# Autodesk Inventor assembly: The_Assembly
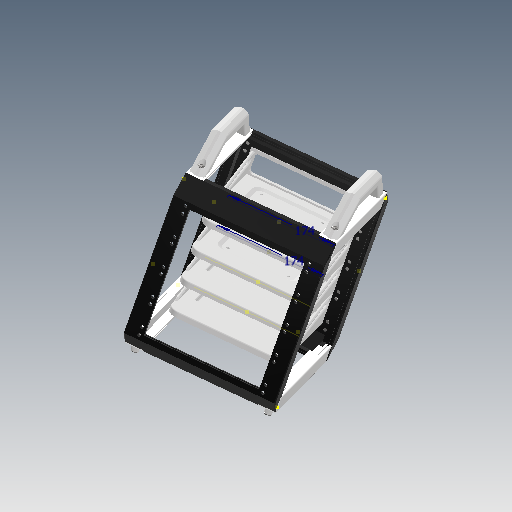
[picture p0: Inventor's stored thumbnail of the model, 512x512]
Saved by Autodesk Inventor 2027 (Build 310192060, 192F)
## iProperties
Created: 2026-07-27
Part Number: The_Assembly
Document SubType Name: Assembly
Designer: prest
Author: prest
## Documents named in this file (24)
- C:\Users\prest\OneDrive\Documents\Projects\Home_Lab_Rack\The_Assembly.iam
- C:\Users\prest\OneDrive\Documents\Projects\Home_Lab_Rack\Strut_Angled.ipt
- C:\Users\prest\OneDrive\Documents\Projects\Home_Lab_Rack\bottom_edge.ipt
- C:\Users\prest\OneDrive\Documents\Projects\Home_Lab_Rack\Strut_Horizontal.ipt
- C:\Users\prest\OneDrive\Documents\Inventor\Content Center Files\R2027\en-US\ANSI B18.3.4M(1)\ANSI B18.3.4M - M6 x 1 x 8(2).ipt
- C:\Users\prest\OneDrive\Documents\Projects\Home_Lab_Rack\mini_PC_mount.ipt
- C:\Users\prest\OneDrive\Documents\Projects\Home_Lab_Rack\router_mount.ipt
- C:\Users\prest\OneDrive\Documents\Projects\Home_Lab_Rack\side_panel_actual.ipt
- C:\Users\prest\OneDrive\Documents\Projects\Home_Lab_Rack\bottom_panel.ipt
- C:\Users\prest\OneDrive\Documents\Projects\Home_Lab_Rack\front_panel_mount_end.ipt
- C:\Users\prest\OneDrive\Documents\Projects\Home_Lab_Rack\top panel.ipt
- C:\Users\prest\OneDrive\Documents\Projects\Home_Lab_Rack\feet.ipt
- C:\Users\prest\OneDrive\Documents\Projects\Home_Lab_Rack\top_edge.ipt
- C:\Users\prest\OneDrive\Documents\Inventor\Content Center Files\R2027\en-US\ASME ANSI B18.3.5M(2)\ASME_ANSI B18.3.5M - M6x20(2).ipt
- C:\Users\prest\OneDrive\Documents\Projects\Home_Lab_Rack\Handle.ipt
- C:\Users\prest\OneDrive\Documents\Inventor\Content Center Files\R2027\en-US\ANSI B18.3.4M(1)\ANSI B18.3.4M - M6 x 1 x 16(2).ipt
- C:\Users\prest\OneDrive\Documents\Projects\Home_Lab_Rack\cable_basket.ipt
- C:\Users\prest\OneDrive\Documents\Projects\Home_Lab_Rack\Strut_Horizonal_Top.ipt
- C:\Users\prest\OneDrive\Documents\Projects\Home_Lab_Rack\MISC\Handle.ipt
- C:\Users\prest\OneDrive\Documents\Projects\Home_Lab_Rack\MISC\Feet.ipt
- C:\Users\prest\OneDrive\Documents\Projects\Home_Lab_Rack\Mounts\Front_Panel_Breathers.ipt
- C:\Users\prest\OneDrive\Documents\Projects\Home_Lab_Rack\Mounts\mini_PC_mount.ipt
- C:\Users\prest\OneDrive\Documents\Projects\Home_Lab_Rack\Mounts\router_mount.ipt
- C:\Users\prest\OneDrive\Documents\Projects\Home_Lab_Rack\Strut_Horizonal_Bottom.ipt
## Components (90 placed, 20 different names)
1. Handle:3 — Rigid:21, Rigid:23, Rigid:26
2. Handle:4 — Rigid:22, Rigid:24, Rigid:25
3. Broached Hexagon Socket Button Head Cap Screw - Metric M6 x 1 x 16:1 — Rigid:23, Rotational:25
4. Broached Hexagon Socket Button Head Cap Screw - Metric M6 x 1 x 16:2 — Rigid:24, Rotational:26
5. Broached Hexagon Socket Button Head Cap Screw - Metric M6 x 1 x 16:3 — Rigid:25, Rotational:27
6. Broached Hexagon Socket Button Head Cap Screw - Metric M6 x 1 x 16:4 — Rigid:26, Rotational:24
7. cable_basket:1 — Rotational:22, Mate:30
8. cable_basket:2 — Rotational:23, Mate:31
9. Strut_Horizonal_Top:1 — Rigid:29, Rigid:30, Rigid:33
10. Strut_Horizonal_Top:2 — Rigid:31, Rigid:32
11. Handle:5 — Rigid:33, Rotational:24, Rotational:26
12. Handle:6 — Rigid:32, Rotational:25, Rotational:27
13. Feet:1 — Rigid:35, Rigid:40
14. Feet:2 — Rigid:36, Rotational:52
15. Feet:3 — Rigid:37, Rigid:39
16. Feet:4 — Rigid:38, Rotational:51
17. Front_Panel_Breathers:1 — Rotational:28, Mate:45, Rotational:39, Rotational:40
18. mini_PC_mount:3 — Mate:39, Mate:40, Mate:41, Rotational:35, Rotational:36, Rotational:43, Rotational:44
19. router_mount:3 — Mate:32, Mate:33, Mate:34, Rotational:31, Rotational:32, Rotational:47, Rotational:48
20. Front_Panel_Breathers:2 — Rotational:29, Mate:35, Rotational:30, Rotational:49
21. router_mount:4 — Mate:36, Mate:37, Mate:38, Rotational:33, Rotational:34, Rotational:45, Rotational:46
22. mini_PC_mount:4 — Mate:42, Mate:43, Mate:44, Rotational:37, Rotational:38, Rotational:41, Rotational:42
23. Broached Hexagon Socket Button Head Cap Screw - Metric M6 x 1 x 16:5 — Rotational:30
24. Broached Hexagon Socket Button Head Cap Screw - Metric M6 x 1 x 16:6 — Rotational:31
25. Broached Hexagon Socket Button Head Cap Screw - Metric M6 x 1 x 16:7 — Rotational:32
26. Broached Hexagon Socket Button Head Cap Screw - Metric M6 x 1 x 16:8 — Rotational:33
27. Broached Hexagon Socket Button Head Cap Screw - Metric M6 x 1 x 16:9 — Rotational:34
28. Broached Hexagon Socket Button Head Cap Screw - Metric M6 x 1 x 16:10 — Rotational:35
29. Broached Hexagon Socket Button Head Cap Screw - Metric M6 x 1 x 16:11 — Rotational:36
30. Broached Hexagon Socket Button Head Cap Screw - Metric M6 x 1 x 16:12 — Rotational:37
31. Broached Hexagon Socket Button Head Cap Screw - Metric M6 x 1 x 16:13 — Rotational:44
32. Broached Hexagon Socket Button Head Cap Screw - Metric M6 x 1 x 16:14 — Rotational:43
33. Broached Hexagon Socket Button Head Cap Screw - Metric M6 x 1 x 16:15 — Rotational:42
34. Broached Hexagon Socket Button Head Cap Screw - Metric M6 x 1 x 16:16 — Rotational:41
35. Broached Hexagon Socket Button Head Cap Screw - Metric M6 x 1 x 16:17 — Rotational:40
36. Broached Hexagon Socket Button Head Cap Screw - Metric M6 x 1 x 16:18 — Rotational:39
37. Broached Hexagon Socket Button Head Cap Screw - Metric M6 x 1 x 16:19 — Rotational:38
38. Broached Hexagon Socket Button Head Cap Screw - Metric M6 x 1 x 16:20 — Rotational:48
39. Broached Hexagon Socket Button Head Cap Screw - Metric M6 x 1 x 16:21 — Rotational:47
40. Broached Hexagon Socket Button Head Cap Screw - Metric M6 x 1 x 16:22 — Rotational:46
41. Broached Hexagon Socket Button Head Cap Screw - Metric M6 x 1 x 16:23 — Rotational:45
42. Broached Hexagon Socket Button Head Cap Screw - Metric M6 x 1 x 16:24 — Rotational:49
43. Strut_Horizonal_Bottom:1 — Rotational:50, Mate:46, Rigid:37, Rigid:38
44. Strut_Horizonal_Bottom:2 — Rigid:34, Rigid:35, Rigid:36
45. Broached Hexagon Socket Flat Countersunk Head Cap Screws - Metric M6x20:5 — Rotational:52
46. Broached Hexagon Socket Flat Countersunk Head Cap Screws - Metric M6x20:6 — Rotational:51
47. Broached Hexagon Socket Flat Countersunk Head Cap Screws - Metric M6x20:3 — Flush:3, Mate:25, Rigid:40
48. Broached Hexagon Socket Flat Countersunk Head Cap Screws - Metric M6x20:4 — Flush:2, Mate:26, Rigid:39
49. Broached Hexagon Socket Button Head Cap Screw - Metric M6 x 1 x 8:1 — Rotational:1
50. Broached Hexagon Socket Button Head Cap Screw - Metric M6 x 1 x 8:2 — Rotational:2
51. Broached Hexagon Socket Button Head Cap Screw - Metric M6 x 1 x 8:3 — Rotational:3
52. Broached Hexagon Socket Button Head Cap Screw - Metric M6 x 1 x 8:4 — Rotational:5
53. Broached Hexagon Socket Button Head Cap Screw - Metric M6 x 1 x 8:5 — Rotational:6
54. Broached Hexagon Socket Button Head Cap Screw - Metric M6 x 1 x 8:6 — Rotational:4
55. Broached Hexagon Socket Button Head Cap Screw - Metric M6 x 1 x 8:7 — Rotational:7
56. Broached Hexagon Socket Button Head Cap Screw - Metric M6 x 1 x 8:8 — Rotational:8
57. Broached Hexagon Socket Button Head Cap Screw - Metric M6 x 1 x 8:13 — Rotational:14
58. Broached Hexagon Socket Button Head Cap Screw - Metric M6 x 1 x 8:14 — Rotational:15
59. Broached Hexagon Socket Button Head Cap Screw - Metric M6 x 1 x 8:15 — Rotational:16
60. Broached Hexagon Socket Button Head Cap Screw - Metric M6 x 1 x 8:17 — Rotational:17
61. Broached Hexagon Socket Button Head Cap Screw - Metric M6 x 1 x 8:18 — Rotational:19
62. Broached Hexagon Socket Button Head Cap Screw - Metric M6 x 1 x 8:19 — Rotational:18
63. Broached Hexagon Socket Button Head Cap Screw - Metric M6 x 1 x 8:20 — Rotational:20
64. Broached Hexagon Socket Button Head Cap Screw - Metric M6 x 1 x 8:21 — Rotational:21
65. Strut_Angled:1 — Rigid:9, Rotational:15, Rotational:16, Rotational:18, Rotational:19, Mate:13, Rigid:16, Mate:19, Mate:20, Mate:22, Mate:24, Rigid:30, Rigid:31
66. Strut_Angled:2 — Rigid:10, Rotational:14, Rotational:17, Rotational:20, Rotational:21, Mate:21, Mate:23, Rigid:29
67. Strut_Angled:3 — Rigid:3, Rigid:4, Rigid:5, Rotational:1, Rotational:2, Rotational:5, Rotational:6, Mate:46, Rigid:34
68. Strut_Angled:4 — Rigid:1, Rigid:2, Rigid:6, Rigid:7, Rotational:3, Rotational:4, Rotational:7, Rotational:8, Mate:16, Rotational:50
69. Strut_Horizontal:1 — Rigid:7, Rigid:9, Mate:1, Mate:2, Mate:4, Mate:5, Mate:8, Mate:11, Mate:14, Mate:17, Rotational:28, Mate:34, Mate:35, Mate:36, Mate:38, Mate:39, Mate:43
70. Strut_Horizontal:2 — Rigid:4, Rotational:22, Rotational:23
71. Strut_Horizontal:3 — Rigid:5, Rigid:10, Mate:30, Mate:31
72. Strut_Horizontal:4 — Rigid:6, Mate:3, Mate:6, Mate:7, Mate:9, Mate:10, Mate:12, Mate:15, Mate:18, Rotational:29, Mate:32, Mate:33, Mate:37, Mate:40, Mate:41, Mate:42, Mate:44, Mate:45
73. bottom_edge:2 — Rigid:1, Rigid:3, Rigid:17, Rigid:18
74. top panel:1 — Rigid:16
75. bottom_edge:3 — Rigid:2, Rigid:15, Rigid:19, Rigid:20
76. top_edge:1 — Mate:22, Mate:23, Mate:24, Rigid:22, Rigid:28
77. top_edge:2 — Mate:19, Mate:20, Mate:21, Rigid:21, Rigid:27
78. feet:1 — Rigid:18
79. feet:2 — Rigid:17
80. feet:3 — Rigid:20, Flush:2, Mate:26
81. feet:4 — Rigid:19, Flush:3, Mate:25
82. mini_PC_mount:1 — Mate:1, Mate:2, Mate:3
83. mini_PC_mount:2 — Mate:4, Mate:5, Mate:6
84. router_mount:1 — Mate:10, Mate:11, Mate:12
85. router_mount:2 — Mate:7, Mate:8, Mate:9
86. side_panel_actual:2 — Rigid:28
87. bottom_panel:1 — Rigid:15
88. side_panel_actual:1 — Rigid:27
89. front_panel_mount_end:2 — Mate:16, Mate:17, Mate:18
90. front_panel_mount_end:1 — Mate:13, Mate:14, Mate:15
## Relationships (127: RevoluteJoint 47, Mate 43, WeldJoint 35, Flush 2)
- Rigid:1 [WeldJoint]: Strut_Angled:4 ↔ bottom_edge:2
- Rigid:2 [WeldJoint]: Strut_Angled:4 ↔ bottom_edge:3
- Rigid:3 [WeldJoint]: Strut_Angled:3 ↔ bottom_edge:2
- Rigid:4 [WeldJoint]: Strut_Angled:3 ↔ Strut_Horizontal:2
- Rigid:5 [WeldJoint]: Strut_Angled:3 ↔ Strut_Horizontal:3
- Rigid:6 [WeldJoint]: Strut_Angled:4 ↔ Strut_Horizontal:4
- Rigid:7 [WeldJoint]: Strut_Angled:4 ↔ Strut_Horizontal:1
- Rotational:1 [RevoluteJoint]: Broached Hexagon Socket Button Head Cap Screw - Metric M6 x 1 x 8:1 ↔ Strut_Angled:3
- Rotational:2 [RevoluteJoint]: Broached Hexagon Socket Button Head Cap Screw - Metric M6 x 1 x 8:2 ↔ Strut_Angled:3
- Rotational:3 [RevoluteJoint]: Broached Hexagon Socket Button Head Cap Screw - Metric M6 x 1 x 8:3 ↔ Strut_Angled:4
- Rotational:4 [RevoluteJoint]: Broached Hexagon Socket Button Head Cap Screw - Metric M6 x 1 x 8:6 ↔ Strut_Angled:4
- Rotational:5 [RevoluteJoint]: Broached Hexagon Socket Button Head Cap Screw - Metric M6 x 1 x 8:4 ↔ Strut_Angled:3
- Rotational:6 [RevoluteJoint]: Broached Hexagon Socket Button Head Cap Screw - Metric M6 x 1 x 8:5 ↔ Strut_Angled:3
- Rotational:7 [RevoluteJoint]: Broached Hexagon Socket Button Head Cap Screw - Metric M6 x 1 x 8:7 ↔ Strut_Angled:4
- Rotational:8 [RevoluteJoint]: Broached Hexagon Socket Button Head Cap Screw - Metric M6 x 1 x 8:8 ↔ Strut_Angled:4
- Rigid:9 [WeldJoint]: Strut_Angled:1 ↔ Strut_Horizontal:1
- Rigid:10 [WeldJoint]: Strut_Angled:2 ↔ Strut_Horizontal:3
- Rotational:14 [RevoluteJoint]: Broached Hexagon Socket Button Head Cap Screw - Metric M6 x 1 x 8:13 ↔ Strut_Angled:2
- Rotational:15 [RevoluteJoint]: Broached Hexagon Socket Button Head Cap Screw - Metric M6 x 1 x 8:14 ↔ Strut_Angled:1
- Rotational:16 [RevoluteJoint]: Broached Hexagon Socket Button Head Cap Screw - Metric M6 x 1 x 8:15 ↔ Strut_Angled:1
- Rotational:17 [RevoluteJoint]: Broached Hexagon Socket Button Head Cap Screw - Metric M6 x 1 x 8:17 ↔ Strut_Angled:2
- Rotational:18 [RevoluteJoint]: Broached Hexagon Socket Button Head Cap Screw - Metric M6 x 1 x 8:19 ↔ Strut_Angled:1
- Rotational:19 [RevoluteJoint]: Broached Hexagon Socket Button Head Cap Screw - Metric M6 x 1 x 8:18 ↔ Strut_Angled:1
- Rotational:20 [RevoluteJoint]: Broached Hexagon Socket Button Head Cap Screw - Metric M6 x 1 x 8:20 ↔ Strut_Angled:2
- Rotational:21 [RevoluteJoint]: Broached Hexagon Socket Button Head Cap Screw - Metric M6 x 1 x 8:21 ↔ Strut_Angled:2
- Rigid:15 [WeldJoint]: bottom_edge:3 ↔ bottom_panel:1
- Mate:1: Strut_Horizontal:1 ↔ mini_PC_mount:1
- Mate:2: Strut_Horizontal:1 ↔ mini_PC_mount:1
- Mate:3: Strut_Horizontal:4 ↔ mini_PC_mount:1
- Mate:4: Strut_Horizontal:1 ↔ mini_PC_mount:2
- Mate:5: Strut_Horizontal:1 ↔ mini_PC_mount:2
- Mate:6: Strut_Horizontal:4 ↔ mini_PC_mount:2
- Mate:7: Strut_Horizontal:4 ↔ router_mount:2
- Mate:8: Strut_Horizontal:1 ↔ router_mount:2
- Mate:9: Strut_Horizontal:4 ↔ router_mount:2
- Mate:10: Strut_Horizontal:4 ↔ router_mount:1
- Mate:11: Strut_Horizontal:1 ↔ router_mount:1
- Mate:12: Strut_Horizontal:4 ↔ router_mount:1
- Mate:13: Strut_Angled:1 ↔ front_panel_mount_end:1
- Mate:14: Strut_Horizontal:1 ↔ front_panel_mount_end:1
- Mate:15: Strut_Horizontal:4 ↔ front_panel_mount_end:1
- Mate:16: Strut_Angled:4 ↔ front_panel_mount_end:2
- Mate:17: Strut_Horizontal:1 ↔ front_panel_mount_end:2
- Mate:18: Strut_Horizontal:4 ↔ front_panel_mount_end:2
- Rigid:16 [WeldJoint]: Strut_Angled:1 ↔ top panel:1
- Rigid:17 [WeldJoint]: bottom_edge:2 ↔ feet:2
- Rigid:18 [WeldJoint]: bottom_edge:2 ↔ feet:1
- Rigid:19 [WeldJoint]: bottom_edge:3 ↔ feet:4
- Rigid:20 [WeldJoint]: bottom_edge:3 ↔ feet:3
- Mate:19: Strut_Angled:1 ↔ top_edge:2
- Mate:20: Strut_Angled:1 ↔ top_edge:2
- Mate:21: Strut_Angled:2 ↔ top_edge:2
- Mate:22: Strut_Angled:1 ↔ top_edge:1
- Mate:23: Strut_Angled:2 ↔ top_edge:1
- Mate:24: Strut_Angled:1 ↔ top_edge:1
- Flush:2 (-1 mm): Broached Hexagon Socket Flat Countersunk Head Cap Screws - Metric M6x20:4 ↔ feet:3
- Flush:3 (-1 mm): Broached Hexagon Socket Flat Countersunk Head Cap Screws - Metric M6x20:3 ↔ feet:4
- Mate:25: Broached Hexagon Socket Flat Countersunk Head Cap Screws - Metric M6x20:3 ↔ feet:4
- Mate:26: Broached Hexagon Socket Flat Countersunk Head Cap Screws - Metric M6x20:4 ↔ feet:3
- Rigid:21 [WeldJoint]: Handle:3 ↔ top_edge:2
- Rigid:22 [WeldJoint]: Handle:4 ↔ top_edge:1
- Rigid:23 [WeldJoint]: Handle:3 ↔ Broached Hexagon Socket Button Head Cap Screw - Metric M6 x 1 x 16:1
- Rigid:24 [WeldJoint]: Handle:4 ↔ Broached Hexagon Socket Button Head Cap Screw - Metric M6 x 1 x 16:2
- Rigid:25 [WeldJoint]: Handle:4 ↔ Broached Hexagon Socket Button Head Cap Screw - Metric M6 x 1 x 16:3
- Rigid:26 [WeldJoint]: Handle:3 ↔ Broached Hexagon Socket Button Head Cap Screw - Metric M6 x 1 x 16:4
- Rigid:27 [WeldJoint]: top_edge:2 ↔ side_panel_actual:1
- Rigid:28 [WeldJoint]: top_edge:1 ↔ side_panel_actual:2
- Rotational:22 [RevoluteJoint]: cable_basket:1 ↔ Strut_Horizontal:2
- Mate:30: cable_basket:1 ↔ Strut_Horizontal:3
- Rotational:23 [RevoluteJoint]: cable_basket:2 ↔ Strut_Horizontal:2
- Mate:31: cable_basket:2 ↔ Strut_Horizontal:3
- Rigid:29 [WeldJoint]: Strut_Horizonal_Top:1 ↔ Strut_Angled:2
- Rigid:30 [WeldJoint]: Strut_Horizonal_Top:1 ↔ Strut_Angled:1
- Rigid:31 [WeldJoint]: Strut_Horizonal_Top:2 ↔ Strut_Angled:1
- Rigid:32 [WeldJoint]: Strut_Horizonal_Top:2 ↔ Handle:6
- Rigid:33 [WeldJoint]: Strut_Horizonal_Top:1 ↔ Handle:5
- Rotational:24 [RevoluteJoint]: Broached Hexagon Socket Button Head Cap Screw - Metric M6 x 1 x 16:4 ↔ Handle:5
- Rotational:25 [RevoluteJoint]: Broached Hexagon Socket Button Head Cap Screw - Metric M6 x 1 x 16:1 ↔ Handle:6
- Rotational:26 [RevoluteJoint]: Broached Hexagon Socket Button Head Cap Screw - Metric M6 x 1 x 16:2 ↔ Handle:5
- Rotational:27 [RevoluteJoint]: Broached Hexagon Socket Button Head Cap Screw - Metric M6 x 1 x 16:3 ↔ Handle:6
- Rotational:28 [RevoluteJoint]: Front_Panel_Breathers:1 ↔ Strut_Horizontal:1
- Rotational:29 [RevoluteJoint]: Front_Panel_Breathers:2 ↔ Strut_Horizontal:4
- Mate:32: router_mount:3 ↔ Strut_Horizontal:4
- Mate:33: router_mount:3 ↔ Strut_Horizontal:4
- Mate:34: router_mount:3 ↔ Strut_Horizontal:1
- Mate:35: Front_Panel_Breathers:2 ↔ Strut_Horizontal:1
- Mate:36: router_mount:4 ↔ Strut_Horizontal:1
- Mate:37: router_mount:4 ↔ Strut_Horizontal:4
- Mate:38: router_mount:4 ↔ Strut_Horizontal:1
- Mate:39: mini_PC_mount:3 ↔ Strut_Horizontal:1
- Mate:40: mini_PC_mount:3 ↔ Strut_Horizontal:4
- Mate:41: mini_PC_mount:3 ↔ Strut_Horizontal:4
- Mate:42: mini_PC_mount:4 ↔ Strut_Horizontal:4
- Mate:43: mini_PC_mount:4 ↔ Strut_Horizontal:1
- Mate:44: mini_PC_mount:4 ↔ Strut_Horizontal:4
- Mate:45: Front_Panel_Breathers:1 ↔ Strut_Horizontal:4
- Rotational:30 [RevoluteJoint]: Front_Panel_Breathers:2 ↔ Broached Hexagon Socket Button Head Cap Screw - Metric M6 x 1 x 16:5
- Rotational:31 [RevoluteJoint]: router_mount:3 ↔ Broached Hexagon Socket Button Head Cap Screw - Metric M6 x 1 x 16:6
- Rotational:32 [RevoluteJoint]: router_mount:3 ↔ Broached Hexagon Socket Button Head Cap Screw - Metric M6 x 1 x 16:7
- Rotational:33 [RevoluteJoint]: router_mount:4 ↔ Broached Hexagon Socket Button Head Cap Screw - Metric M6 x 1 x 16:8
- Rotational:34 [RevoluteJoint]: router_mount:4 ↔ Broached Hexagon Socket Button Head Cap Screw - Metric M6 x 1 x 16:9
- Rotational:35 [RevoluteJoint]: mini_PC_mount:3 ↔ Broached Hexagon Socket Button Head Cap Screw - Metric M6 x 1 x 16:10
- Rotational:36 [RevoluteJoint]: mini_PC_mount:3 ↔ Broached Hexagon Socket Button Head Cap Screw - Metric M6 x 1 x 16:11
- Rotational:37 [RevoluteJoint]: mini_PC_mount:4 ↔ Broached Hexagon Socket Button Head Cap Screw - Metric M6 x 1 x 16:12
- Rotational:38 [RevoluteJoint]: mini_PC_mount:4 ↔ Broached Hexagon Socket Button Head Cap Screw - Metric M6 x 1 x 16:19
- Rotational:39 [RevoluteJoint]: Front_Panel_Breathers:1 ↔ Broached Hexagon Socket Button Head Cap Screw - Metric M6 x 1 x 16:18
- Rotational:40 [RevoluteJoint]: Front_Panel_Breathers:1 ↔ Broached Hexagon Socket Button Head Cap Screw - Metric M6 x 1 x 16:17
- Rotational:41 [RevoluteJoint]: mini_PC_mount:4 ↔ Broached Hexagon Socket Button Head Cap Screw - Metric M6 x 1 x 16:16
- Rotational:42 [RevoluteJoint]: mini_PC_mount:4 ↔ Broached Hexagon Socket Button Head Cap Screw - Metric M6 x 1 x 16:15
- Rotational:43 [RevoluteJoint]: mini_PC_mount:3 ↔ Broached Hexagon Socket Button Head Cap Screw - Metric M6 x 1 x 16:14
- Rotational:44 [RevoluteJoint]: mini_PC_mount:3 ↔ Broached Hexagon Socket Button Head Cap Screw - Metric M6 x 1 x 16:13
- Rotational:45 [RevoluteJoint]: router_mount:4 ↔ Broached Hexagon Socket Button Head Cap Screw - Metric M6 x 1 x 16:23
- Rotational:46 [RevoluteJoint]: router_mount:4 ↔ Broached Hexagon Socket Button Head Cap Screw - Metric M6 x 1 x 16:22
- Rotational:47 [RevoluteJoint]: router_mount:3 ↔ Broached Hexagon Socket Button Head Cap Screw - Metric M6 x 1 x 16:21
- Rotational:48 [RevoluteJoint]: router_mount:3 ↔ Broached Hexagon Socket Button Head Cap Screw - Metric M6 x 1 x 16:20
- Rotational:49 [RevoluteJoint]: Front_Panel_Breathers:2 ↔ Broached Hexagon Socket Button Head Cap Screw - Metric M6 x 1 x 16:24
- Rotational:50 [RevoluteJoint]: Strut_Horizonal_Bottom:1 ↔ Strut_Angled:4
- Mate:46: Strut_Horizonal_Bottom:1 ↔ Strut_Angled:3
- Rigid:34 [WeldJoint]: Strut_Horizonal_Bottom:2 ↔ Strut_Angled:3
- Rigid:35 [WeldJoint]: Feet:1 ↔ Strut_Horizonal_Bottom:2
- Rigid:36 [WeldJoint]: Feet:2 ↔ Strut_Horizonal_Bottom:2
- Rigid:37 [WeldJoint]: Feet:3 ↔ Strut_Horizonal_Bottom:1
- Rigid:38 [WeldJoint]: Feet:4 ↔ Strut_Horizonal_Bottom:1
- Rigid:39 [WeldJoint]: Feet:3 ↔ Broached Hexagon Socket Flat Countersunk Head Cap Screws - Metric M6x20:4
- Rigid:40 [WeldJoint]: Feet:1 ↔ Broached Hexagon Socket Flat Countersunk Head Cap Screws - Metric M6x20:3
- Rotational:51 [RevoluteJoint]: Feet:4 ↔ Broached Hexagon Socket Flat Countersunk Head Cap Screws - Metric M6x20:6
- Rotational:52 [RevoluteJoint]: Feet:2 ↔ Broached Hexagon Socket Flat Countersunk Head Cap Screws - Metric M6x20:5
